# Autodesk Inventor assembly: sholder
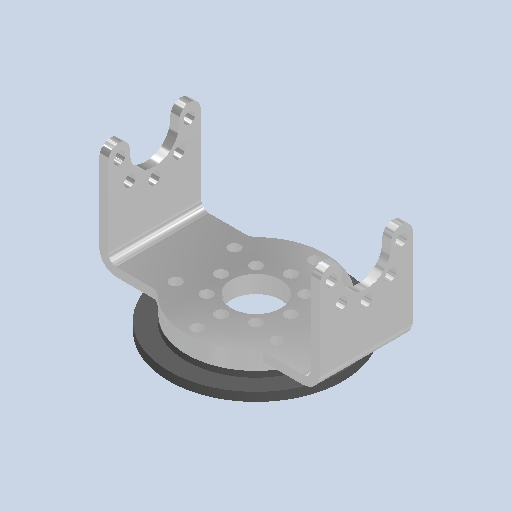
[picture p0: Inventor's stored thumbnail of the model, 512x512]
Saved by Autodesk Inventor 2024.1 (Build 281209000, 209)
## iProperties
Created: 2024-02-14
Part Number: sholder
Document SubType Name: Assembly
Designer: hibik
Author: hibik
## Documents named in this file (4)
- C:\Users\hibik\Desktop\ロボメカ\HR\2024.02.11 Rl\02.11 ProtType\sholder.iam
- C:\Users\hibik\Desktop\ロボメカ\HR\2024.02.11 Rl\02.11 ProtType\sholder.ipt
- C:\Users\hibik\Desktop\ロボメカ\HR\2024.02.11 Rl\02.11 ProtType\sholder_joint_s.ipt
- C:\Users\hibik\Desktop\ロボメカ\HR\2024.02.11 Rl\02.11 ProtType\sholder_joint_c.ipt
## Components (3 placed, 3 different names)
1. sholder:1 — 挿入:1, 挿入:3
2. sholder_joint_s:1 — 挿入:1, 挿入:3, 挿入:4, 挿入:5
3. sholder_joint_c:1 — 挿入:4, 挿入:5
## Relationships (4: Insert 4)
- 挿入:1 [Insert]: sholder:1 ↔ sholder_joint_s:1
- 挿入:3 [Insert]: sholder:1 ↔ sholder_joint_s:1
- 挿入:4 [Insert]: sholder_joint_s:1 ↔ sholder_joint_c:1
- 挿入:5 [Insert]: sholder_joint_s:1 ↔ sholder_joint_c:1
